# Autodesk Inventor assembly: Motor_MIR1
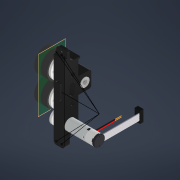
[picture p0: Inventor's stored thumbnail of the model, 180x180]
Saved by Autodesk Inventor 2022 (Build 260153000, 153)
## iProperties
Created: 2021-09-24
Part Number: Motor_MIR1
Document SubType Name: Assembly
Designer: shiok
Mass: 25.2462 g
Surface Area: 225.449 cm^2
Volume: 18.4581 cm^3
Density: 1.36776 g/cm^3
Author: shiok
## Documents named in this file (7)
- C:\Users\shiok\Documents\GitHub\murakumo\inventor\Motor_MIR1.iam
- C:\Users\shiok\Documents\GitHub\murakumo\inventor\MotorBracket_MIR3.ipt
- C:\Users\shiok\Documents\GitHub\murakumo\inventor\maxon DCX 10L_MIR3.iam
- C:\Users\shiok\Documents\GitHub\murakumo\inventor\Tire_MIR3.iam
- C:\Users\shiok\Documents\GitHub\murakumo\inventor\FL674ZZ_MIR3.ipt
- C:\Users\shiok\Documents\GitHub\murakumo\inventor\piniongear_41_middle_MIR3.ipt
- C:\Users\shiok\Documents\GitHub\murakumo\inventor\piniongear_41_src_MIR3.ipt
## Components (8 placed, 6 different names)
1. MotorBracket_MIR3:1 — メイト:14, メイト:13, メイト:7, フラッシュ:4, フラッシュ:1, メイト:5, フラッシュ:3, メイト:6, フラッシュ:2, メイト:4, メイト:3, メイト:2, メイト:1
2. maxon DCX 10L_MIR3:1 [sub-assembly] — メイト:14, メイト:13, メイト:7, メイト:12
3. Tire_MIR3:1 [sub-assembly] — フラッシュ:4, フラッシュ:1, メイト:5, フラッシュ:7, 対称度:1
4. Tire_MIR3:2 [sub-assembly] — フラッシュ:3, メイト:6, フラッシュ:2, 対称度:1
5. FL674ZZ_MIR3:1 — メイト:4, メイト:3
6. FL674ZZ_MIR3:2 — メイト:2, メイト:1
7. piniongear_41_middle_MIR3:1
8. piniongear_41_src_MIR3:1 — フラッシュ:7, メイト:12
## Relationships (16: Mate 10, Flush 5, Symmetry 1)
- メイト:14 [Mate]: MotorBracket_MIR3:1 ↔ maxon DCX 10L_MIR3:1
- メイト:13 [Mate]: MotorBracket_MIR3:1 ↔ maxon DCX 10L_MIR3:1
- メイト:7 [Mate]: MotorBracket_MIR3:1 ↔ maxon DCX 10L_MIR3:1
- フラッシュ:4 [Flush]: MotorBracket_MIR3:1 ↔ Tire_MIR3:1
- フラッシュ:1 [Flush]: MotorBracket_MIR3:1 ↔ Tire_MIR3:1
- メイト:5 [Mate]: MotorBracket_MIR3:1 ↔ Tire_MIR3:1
- フラッシュ:3 [Flush]: MotorBracket_MIR3:1 ↔ Tire_MIR3:2
- メイト:6 [Mate]: MotorBracket_MIR3:1 ↔ Tire_MIR3:2
- フラッシュ:2 [Flush]: MotorBracket_MIR3:1 ↔ Tire_MIR3:2
- メイト:4 [Mate]: MotorBracket_MIR3:1 ↔ FL674ZZ_MIR3:1
- メイト:3 [Mate]: MotorBracket_MIR3:1 ↔ FL674ZZ_MIR3:1
- メイト:2 [Mate]: MotorBracket_MIR3:1 ↔ FL674ZZ_MIR3:2
- メイト:1 [Mate]: MotorBracket_MIR3:1 ↔ FL674ZZ_MIR3:2
- フラッシュ:7 [Flush]: Tire_MIR3:1 ↔ piniongear_41_src_MIR3:1
- メイト:12 [Mate]: maxon DCX 10L_MIR3:1 ↔ piniongear_41_src_MIR3:1
- 対称度:1 [Symmetry]: Tire_MIR3:1 ↔ Tire_MIR3:2
